# Autodesk Inventor assembly: NR-025.5-D(F,D-770)
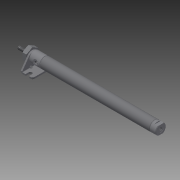
[picture p0: Inventor's stored thumbnail of the model, 180x180]
Saved by Autodesk Inventor 2013 (Build 170138000, 138)
## iProperties
Created: 2013-01-26
Part Number: NR-025.5-D(F,D-770)
Catalog Web Link: www.cadenas.de
Description: Non-Rotating Original Line Air Cylinder-
Vendor: BIMBA
Document SubType Name: Assembly
Designer: actoennies
Manufacturer: BIMBA
Category: PARTsolutions
Company: BIMBA
Title: NR-025.5-D
Author: Cadenas PARTsolutions
PSOL_IDENT_0: {\\10.0.0.242\data_v9\23d-libs\bimba\bimba\bimba_imperial\bimba_full_line\original_line_cylinders\no
PSOL_IDENT_1: n_rotating_air_cylinders\nr_cylinder_asmtab.prj},290 {VTYP=3D},{STYP=ASSTAB},{NB=NR-025.5-D(F,D-770)
PSOL_IDENT_2: },{LINA=NR-025.5-D},{NN=Non-Rotating Original Line Air Cylinder},{DATE=13.06.2012 09:03:04},{GEOMDAT
PSOL_IDENT_3: E=13.06.2012},{VERSION=},{LINEID=40},{LINESUBID=-1},{WBVAR=STROKE,ACTING,MNT,M,NT,EE,EEL,G,K,Q,Y,B,T
PSOL_IDENT_4: ,STPT1,STPT2,STPT3,STPT4,MB,MN,PB,PRC,TB}  {NB=NR-025.5-D(F,D-770)},{LINA=NR-025.5-D},{KT=DUMMY},{PN
PSOL_IDENT_5: =NR-025.5-D},{PNC=NR-025.5-D(F,D-770)},{PNA=(D-770)},{DASH=-},{BORE=9/16\" (02)},{BORE1=0.56250000},
PSOL_IDENT_6: {BOREPN=02},{STROKE=5.500},{STROKEALG=[0.011:50/0.001]},{STROKE1=5.500},{ACTING=D},{ACTINGALG= 'R' ,
PSOL_IDENT_7: 'Reverse Single Acting (NR)' , 'D' , 'Double Acting (NR)'  ,'DXDE','Double Ended Rod (NR)'},{ACTING
PSOL_IDENT_8: PN=D},{MNT=},{MNTALG= '' , 'Front Nose Mounting (NR)' , 'XP' , 'Double End or Rear Pivot Mounting (N
PSOL_IDENT_9: R)' },{TYPE=NR-},{MNTPN=},{NR=},{NRALG= '' , 'N/A' },{NRPN=},{BM=},{BMALG= '' , 'N/A' },{BMPN=},{CO=
PSOL_IDENT_10: },{COALG= '' , 'N/A' },{OO=},{OOALG= '', 'N/A' },{OOPN=},{VO=},{VOALG= 'Z' , 'N/A' },{VOPN=},{DER=},
PSOL_IDENT_11: {DERALG= '' , 'N/A' },{F=},{FALG= '', 'Non-Coated (Standard)', 'F', 'Molycoated' },{FPN=},{SR=},{SRA
PSOL_IDENT_12: LG= '' , '303 Stainless Steel Rod' },{SRPN=},{M=},{MALG= '', 'W/out Magnet', 'M', 'W/ Magnet' },{NT=
PSOL_IDENT_13: },{NTPN=},{EE=},{EEL=0.000},{EEMAX=44.5000},{EEALG= '', 'W/out Extra Extension', 'EE', 'W/ Extra Ext
PSOL_IDENT_14: ension' },{EELALG=0},{EEPN=},{EEPN1=0.000},{G=},{GPN=},{GPN1=},{K=},{KALG= '' , 'N/A' },{KPN=},{Q=},
PSOL_IDENT_15: {QALG= '' , 'Standard Port' , 'Q' , 'Side Port' },{QPN=},{Y=},{YALG= '' , 'N/A' },{YPN=},{YCON=},{B=
PSOL_IDENT_16: },{BALG= '', 'W/out Bumper' , 'B' , 'W/ Bumper' },{BPN=},{H=},{HALG= '', 'N/A' },{HPN=},{T=},{TALG=
PSOL_IDENT_17: '' , 'Standard -20° to 200°F (-29° to 95°C)' , 'N' , 'Low Temperature' , 'V' , 'High Temperature' },
PSOL_IDENT_18: {NPN=},{VPN=},{W=},{WALG= '' , 'W/out Wiper' , 'W' , 'W/ Wiper' },{WPN=},{E=},{EALG= '' , 'Standard
PSOL_IDENT_19: Seals/Lube' , 'E' , 'Non-Lube Seals/Lube' },{EPN=},{HL=},{HLALG= '' , 'W/out Low Pressure Hydraulic'
PSOL_IDENT_20: , 'HL' , 'W/ Low Pressure Hydraulic' },{ST=},{STALG= '' , 'N/A' },{STPT1=},{STPT1ALG= '' , 'N/A' },
PSOL_IDENT_21: {STPT1PN=},{STPT2=},{STPT2ALG= '' , 'N/A' },{STPT3=},{STPT3ALG= '' , 'N/A' },{STPT4=},{STPT4ALG= ''
PSOL_IDENT_22: , 'N/A' },{STPN=},{SER=},{SERALG= '' , 'W/out Spring Extend/Return' , 'JS' , 'W/ Spring Return' , 'J
PSOL_IDENT_23: R' , 'W/ Spring Extend' },{MB=F,D-770},{MBALG= '' , 'W/out Mounting Bracket' , 'F,D-770' , 'D-770 (f
PSOL_IDENT_24: ront)' },{MBPN=(F,D-770)},{MBPNALL=D-770},{MN=},{MNALG= '' , 'N/A' },{MNPN=},{PB=},{PBALG= '' , 'N/A
PSOL_IDENT_25: ' },{PBPN=},{PBPNALL=},{PRC=},{PRCALG= '' , 'N/A' },{PRCPN=},{PRCPNALL=},{TB=},{TBALG= '' , 'N/A' },
PSOL_IDENT_26: {TBPN=},{TBPNALL=},{SPACE=0.0763},{TEXT=0.1336},{FNUTPN=D-154},{RNUTPN=},{AALG=2.28},{A=2.28},{A1ALG
PSOL_IDENT_27: =0.00},{A1=-},{AA=-},{AAALG=0.00},{AA1=-},{DALG=0.50},{D=0.5},{O=#10-32},{N=0.22},{M1=7/16-20},{L=.4
PSOL_IDENT_28: 34/.437},{F1=#10-32},{H1=0.62},{C=0.75},{B1=0.38},{G1=0.19},{K1=0.50},{E1=0.06},{P=-},{Q1=-},{R1=-},
PSOL_IDENT_29: {S1=-},{V1=-},{W1=-},{W11=-},{L1=-},{Z=-},{Y1=-},{Y11=-},{MBR=},{MBF=F},{MNF=},{MNR=},{FNUTCON=1},{F
PSOL_IDENT_30: NUTCON1=0},{RNUTCON=0},{RNUTCON1=0},{MATALGHTML=<b>Non-Rotating Original Line Cylinder:</b><dl><dt>R
PSOL_IDENT_31: od:</dt><dd>- 304 Stainless Steel</dd><dt>Bearings:</dt><dd>- Aluminum </dd><dt>Body:</dt><dd>- 304
PSOL_IDENT_32: Stainless Steel</dd><dt>End Caps:</dt><dd>- Aluminum</dd><dt>Seals:</dt><dd>-  Buna N</dd></dl>},{PP
PSOL_IDENT_33: ATH=nr_cylinder_asmtpl.prj},{MBP=(D-770)},{MNP=},{PRCP=},{ASSOPTACC=STPT4},{DIF=0.00}
CNS_NT: Standard Male Thread
CNS_NB: NR-025.5-D(F,D-770)
CNS_NBSYN: $PNC.
CNS_LINA: NR-025.5-D
CNS_PN: NR-025.5-D
CNS_PNC: NR-025.5-D(F,D-770)
CNS_PNA: (D-770)
CNS_DASH: -
CNS_BORE: 9/16" [02]
CNS_BORE1: 0.56250000
CNS_BOREPN: 02
CNS_STROKE: 5.500
CNS_STROKEALG: [0.011:50/0.001]
CNS_STROKE1: 5.500
CNS_ACTING: Double [D]
CNS_ACTINGALG: 'R' , 'Reverse Single Acting (NR)' , 'D' , 'Double Acting (NR)'  ,'DXDE','Double Ended Rod (NR)'
CNS_ACTINGPN: D
CNS_MNT: Standard Front Nose
CNS_MNTALG: '' , 'Front Nose Mounting (NR)' , 'XP' , 'Double End or Rear Pivot Mounting (NR)'
CNS_TYPE: NR-
CNS_NRALG: '' , 'N/A'
CNS_BMALG: '' , 'N/A'
CNS_COALG: '' , 'N/A'
CNS_OOALG: '', 'N/A'
CNS_VOALG: 'Z' , 'N/A'
CNS_DERALG: '' , 'N/A'
CNS_FALG: '', 'Non-Coated (Standard)', 'F', 'Molycoated'
CNS_SRALG: '' , '303 Stainless Steel Rod'
CNS_M: Standard Non-Magnetic Piston
CNS_MALG: '', 'W/out Magnet', 'M', 'W/ Magnet'
CNS_EE: Standard Rod Extension
CNS_EEL: 0.000
CNS_EEMAX: 44.5000
CNS_EEALG: '', 'W/out Extra Extension', 'EE', 'W/ Extra Extension'
CNS_EELALG: 0
CNS_EEPN1: 0.000
CNS_G: Standard Grease Lube
CNS_K: N/A
CNS_KALG: '' , 'N/A'
CNS_Q: Standard Axial Port
CNS_QALG: '' , 'Standard Port' , 'Q' , 'Side Port'
CNS_Y: N/A
CNS_YALG: '' , 'N/A'
CNS_B: Without Bumpers
CNS_BALG: '', 'W/out Bumper' , 'B' , 'W/ Bumper'
CNS_HALG: '', 'N/A'
CNS_T: Standard -20° to 200°F (-29° to 95°C)
CNS_TALG: '' , 'Standard -20° to 200°F (-29° to 95°C)' , 'N' , 'Low Temperature' , 'V' , 'High Temperature'
CNS_WALG: '' , 'W/out Wiper' , 'W' , 'W/ Wiper'
CNS_EALG: '' , 'Standard Seals/Lube' , 'E' , 'Non-Lube Seals/Lube'
CNS_HLALG: '' , 'W/out Low Pressure Hydraulic' , 'HL' , 'W/ Low Pressure Hydraulic'
CNS_STALG: '' , 'N/A'
CNS_STPT1: N/A
CNS_STPT1ALG: '' , 'N/A'
CNS_STPT2: N/A
CNS_STPT2ALG: '' , 'N/A'
CNS_STPT3: N/A
CNS_STPT3ALG: '' , 'N/A'
CNS_STPT4: N/A
CNS_STPT4ALG: '' , 'N/A'
CNS_SERALG: '' , 'W/out Spring Extend/Return' , 'JS' , 'W/ Spring Return' , 'JR' , 'W/ Spring Extend'
CNS_MB: D-770 (front)
CNS_MBALG: '' , 'W/out Mounting Bracket' , 'F,D-770' , 'D-770 (front)'
CNS_MBPN: (F,D-770)
CNS_MBPNALL: D-770
CNS_MN: N/A
CNS_MNALG: '' , 'N/A'
CNS_PB: N/A
CNS_PBALG: '' , 'N/A'
CNS_PRC: N/A
CNS_PRCALG: '' , 'N/A'
CNS_TB: N/A
CNS_TBALG: '' , 'N/A'
CNS_SPACE: 0.0763
CNS_TEXT: 0.1336
CNS_FNUTPN: D-154
CNS_AALG: 2.28
CNS_A: 2.28
CNS_A1ALG: 0.00
CNS_A1: -
CNS_AA: -
CNS_AAALG: 0.00
CNS_AA1: -
CNS_DALG: 0.50
CNS_D: 0.5
CNS_O: #10-32
CNS_N: 0.22
CNS_M1: 7/16-20
CNS_L: .434/.437
CNS_F1: #10-32
CNS_H1: 0.62
CNS_C: 0.75
CNS_B1: 0.38
CNS_G1: 0.19
CNS_K1: 0.50
CNS_E1: 0.06
CNS_P: -
CNS_Q1: -
CNS_R1: -
CNS_S1: -
CNS_V1: -
CNS_W1: -
CNS_W11: -
CNS_L1: -
CNS_Z: -
CNS_Y1: -
CNS_Y11: -
CNS_MBF: F
CNS_FNUTCON: 1
CNS_FNUTCON1: 0
CNS_RNUTCON: 0
CNS_RNUTCON1: 0
CNS_MATALGHTML: <b>Non-Rotating Original Line Cylinder:</b><dl><dt>Rod:</dt><dd>- 304 Stainless Steel</dd><dt>Bearings:</dt><dd>- Aluminum </dd><dt>Body:</dt><dd>- 304 Stainless Steel</dd><dt>End Caps:</dt><dd>- Aluminum</dd><dt>Seals:</dt><dd>-  Buna N</dd></dl>
CNS_PPATH: nr_cylinder_asmtpl.prj
CNS_MBP: (D-770)
CNS_ASSOPTACC: STPT4
CNS_DIF: 0.00
SUPPLIER: BIMBA
ARTICLENO: NR-025.5-D(F,D-770)
BOMINFO: NR-025.5-D
CREATOR: CADENAS GmbH
## Documents named in this file (7)
- \\NNHSSRV2.hs.sd203.org\ACToennies$\Robotics\Parts\NR-025_5-D(F,D-770).iam
- \\NNHSSRV2.hs.sd203.org\ACToennies$\Robotics\Parts\02R0101_NR_rod_guide.ipt
- \\NNHSSRV2.hs.sd203.org\ACToennies$\Robotics\Parts\025_5-D_NR_rod.ipt
- \\NNHSSRV2.hs.sd203.org\ACToennies$\Robotics\Parts\02-6_3880-nr.ipt
- \\NNHSSRV2.hs.sd203.org\ACToennies$\Robotics\Parts\02R00_NR_rear_head.ipt
- \\NNHSSRV2.hs.sd203.org\ACToennies$\Robotics\Parts\D-154.ipt
- \\NNHSSRV2.hs.sd203.org\ACToennies$\Robotics\Parts\D-770.ipt
## Components (6 placed, 6 different names)
1. 02R0101_NR_rod_guide:1 — rod_guide_Z@1 <-> rod_cp_Z@2, rod_guide_YZ@1 <-> rod_cp_YZ@2, to_tube_XY@1 <-> tube_front_XY@3, to_tube_Z@1 <-> tube_front_Z@3, to_tube_YZ@1 <-> tube_front_YZ@3, to_nut_XY@1 <-> NUT_XY@5, to_nut_Z@1 <-> NUT_Z@5, to_nut_XY@1 <-> mounting_bracket_XY@6, to_nut_Z@1 <-> mounting_bracket_Z@6
2. 025_5-D_NR_rod:1 — rod_guide_Z@1 <-> rod_cp_Z@2, rod_guide_YZ@1 <-> rod_cp_YZ@2
3. 02-6_3880-nr:1 — to_tube_XY@1 <-> tube_front_XY@3, to_tube_Z@1 <-> tube_front_Z@3, to_tube_YZ@1 <-> tube_front_YZ@3, tube_rear_XY@3 <-> to_tube_XY@4, tube_rear_Z@3 <-> to_tube_Z@4, tube_rear_YZ@3 <-> to_tube_YZ@4
4. 02R00_NR_rear_head:1 — tube_rear_XY@3 <-> to_tube_XY@4, tube_rear_Z@3 <-> to_tube_Z@4, tube_rear_YZ@3 <-> to_tube_YZ@4
5. D-154:1 — to_nut_XY@1 <-> NUT_XY@5, to_nut_Z@1 <-> NUT_Z@5
6. D-770:1 — to_nut_XY@1 <-> mounting_bracket_XY@6, to_nut_Z@1 <-> mounting_bracket_Z@6
## Relationships (12: Mate 5, Flush 4, Angle 3)
- rod_guide_Z@1 <-> rod_cp_Z@2 [Mate]: 02R0101_NR_rod_guide:1 ↔ 025_5-D_NR_rod:1
- rod_guide_YZ@1 <-> rod_cp_YZ@2 [Angle] (0 deg): 02R0101_NR_rod_guide:1 ↔ 025_5-D_NR_rod:1
- to_tube_XY@1 <-> tube_front_XY@3 [Flush]: 02R0101_NR_rod_guide:1 ↔ 02-6_3880-nr:1
- to_tube_Z@1 <-> tube_front_Z@3 [Mate]: 02R0101_NR_rod_guide:1 ↔ 02-6_3880-nr:1
- to_tube_YZ@1 <-> tube_front_YZ@3 [Angle] (0 deg): 02R0101_NR_rod_guide:1 ↔ 02-6_3880-nr:1
- tube_rear_XY@3 <-> to_tube_XY@4 [Flush]: 02-6_3880-nr:1 ↔ 02R00_NR_rear_head:1
- tube_rear_Z@3 <-> to_tube_Z@4 [Mate]: 02-6_3880-nr:1 ↔ 02R00_NR_rear_head:1
- tube_rear_YZ@3 <-> to_tube_YZ@4 [Angle] (0 deg): 02-6_3880-nr:1 ↔ 02R00_NR_rear_head:1
- to_nut_XY@1 <-> NUT_XY@5 [Flush] (-2.2784 mm): 02R0101_NR_rod_guide:1 ↔ D-154:1
- to_nut_Z@1 <-> NUT_Z@5 [Mate]: 02R0101_NR_rod_guide:1 ↔ D-154:1
- to_nut_XY@1 <-> mounting_bracket_XY@6 [Flush]: 02R0101_NR_rod_guide:1 ↔ D-770:1
- to_nut_Z@1 <-> mounting_bracket_Z@6 [Mate]: 02R0101_NR_rod_guide:1 ↔ D-770:1
